# Autodesk Inventor assembly: RotatingPart
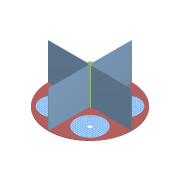
[picture p0: Inventor's stored thumbnail of the model, 180x180]
Saved by Autodesk Inventor 2018 (Build 220112000, 112)
## iProperties
Created: 2017-12-09
Part Number: RotatingPart
Document SubType Name: Assembly
Designer: Udara Wanasinghe
Author: Udara Wanasinghe
## Documents named in this file (4)
- D:\Documents\FIT\Hardware Project\Perfect\RotatingPart.iam
- D:\Documents\FIT\Hardware Project\Perfect\Plate.ipt
- D:\Documents\FIT\Hardware Project\Perfect\MeshPlate.ipt
- D:\Documents\FIT\Hardware Project\Perfect\4PlatesNMiddleShaft.iam
## Components (6 placed, 3 different names)
1. Plate:1 — Rigid:1, Rigid:2, Rigid:3, Rigid:4, Rigid:5
2. MeshPlate:1 — Rigid:1
3. MeshPlate:2 — Rigid:2
4. MeshPlate:3 — Rigid:3
5. MeshPlate:4 — Rigid:4
6. 4PlatesNMiddleShaft:1 [sub-assembly] — Rigid:5
## Relationships (5: WeldJoint 5)
- Rigid:1 [WeldJoint]: Plate:1 ↔ MeshPlate:1
- Rigid:2 [WeldJoint]: Plate:1 ↔ MeshPlate:2
- Rigid:3 [WeldJoint]: Plate:1 ↔ MeshPlate:3
- Rigid:4 [WeldJoint]: Plate:1 ↔ MeshPlate:4
- Rigid:5 [WeldJoint]: Plate:1 ↔ 4PlatesNMiddleShaft:1
